# Autodesk Inventor assembly: FemPodstawa
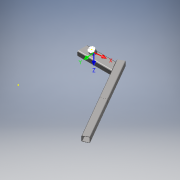
[picture p0: Inventor's stored thumbnail of the model, 180x180]
Saved by Autodesk Inventor 2017 (Build 210142000, 142)
## iProperties
Created: 2016-12-08
Part Number: FemPodstawa
Document SubType Name: Assembly
Designer: Marcin
Author: Marcin
## Documents named in this file (21)
- M:\PracaInżynierska\FEM\FemPodstawa.iam
- M:\PracaInżynierska\PodstawaFem.ipt
- M:\PracaInżynierska\WynikiZadaniaOdwrotnego\PN EN 10219-2 - 100 x 80 x 6  - 655.ipt
- M:\PracaInżynierska\WynikiZadaniaOdwrotnego\PN EN 10219-2 - 160 x 80 x 8  - 545.ipt
- M:\PracaInżynierska\WynikiZadaniaOdwrotnego\PN EN 10060 - 75 - 50.ipt
- M:\PracaInżynierska\WynikiZadaniaOdwrotnego\PN EN 10219-2 - 100 x 80 x 6  - 655_MIR.ipt
- M:\PracaInżynierska\WynikiZadaniaOdwrotnego\PN EN 10219-2 - 160 x 80 x 8  - 545_MIR.ipt
- M:\PracaInżynierska\WynikiZadaniaOdwrotnego\PN EN 10060 - 75 - 50_MIR.ipt
- M:\PracaInżynierska\WynikiZadaniaOdwrotnego\PN EN 10219-2 - 100 x 80 x 6  - 655_MIR1.ipt
- M:\PracaInżynierska\WynikiZadaniaOdwrotnego\PN EN 10219-2 - 160 x 80 x 8  - 545_MIR1.ipt
- M:\PracaInżynierska\WynikiZadaniaOdwrotnego\PN EN 10060 - 75 - 50_MIR1.ipt
- M:\PracaInżynierska\WynikiZadaniaOdwrotnego\PN EN 10219-2 - 100 x 80 x 6  - 655_MIR_MIR.ipt
- M:\PracaInżynierska\WynikiZadaniaOdwrotnego\PN EN 10219-2 - 160 x 80 x 8  - 545_MIR_MIR.ipt
- M:\PracaInżynierska\WynikiZadaniaOdwrotnego\PN EN 10060 - 75 - 50_MIR_MIR.ipt
- M:\PracaInżynierska\PodstawaFem_MIR.ipt
- M:\PracaInżynierska\WynikiZadaniaOdwrotnego\PN EN 10219-2 - 100 x 80 x 6  - 655_MIR2.ipt
- M:\PracaInżynierska\WynikiZadaniaOdwrotnego\PN EN 10219-2 - 160 x 80 x 8  - 545_MIR2.ipt
- M:\PracaInżynierska\WynikiZadaniaOdwrotnego\PN EN 10060 - 75 - 50_MIR2.ipt
- M:\PracaInżynierska\WynikiZadaniaOdwrotnego\PN EN 10219-2 - 100 x 80 x 6  - 655_MIR_MIR1.ipt
- M:\PracaInżynierska\WynikiZadaniaOdwrotnego\PN EN 10219-2 - 160 x 80 x 8  - 545_MIR_MIR1.ipt
- M:\PracaInżynierska\WynikiZadaniaOdwrotnego\PN EN 10060 - 75 - 50_MIR_MIR1.ipt
## Components (20 placed, 20 different names)
1. PodstawaFem:1 — Flush:13
2. PN EN 10219-2 - 100 x 80 x 6  - 655:1 — Mate:3, Flush:5
3. PN EN 10219-2 - 160 x 80 x 8  - 545:1 — Mate:3, Flush:5, Mate:4
4. PodSilownik — Mate:4, Flush:13
5. PN EN 10219-2 - 100 x 80 x 6  - 655_MIR:1 — Flush:6, Mate:5
6. PN EN 10219-2 - 160 x 80 x 8  - 545_MIR:1 — Flush:6, Mate:5, Angle:2, Mate:6
7. PN EN 10060 - 75 - 50_MIR:1 — Angle:2, Mate:6
8. PN EN 10219-2 - 100 x 80 x 6  - 655_MIR1:1 — Flush:7, Mate:7
9. PN EN 10219-2 - 160 x 80 x 8  - 545_MIR1:1 — Flush:7, Mate:7, Angle:3, Mate:8
10. PN EN 10060 - 75 - 50_MIR1:1 — Angle:3, Mate:8
11. PN EN 10219-2 - 100 x 80 x 6  - 655_MIR_MIR:1 — Mate:9, Flush:8
12. PN EN 10219-2 - 160 x 80 x 8  - 545_MIR_MIR:1 — Mate:9, Flush:8, Mate:10, Angle:4
13. PN EN 10060 - 75 - 50_MIR_MIR:1 — Mate:10, Angle:4
14. PodstawaFem_MIR:1
15. PN EN 10219-2 - 100 x 80 x 6  - 655_MIR2:1 — Flush:9, Mate:11
16. PN EN 10219-2 - 160 x 80 x 8  - 545_MIR2:1 — Flush:9, Mate:11, Angle:5, Mate:12
17. PN EN 10060 - 75 - 50_MIR2:1 — Angle:5, Mate:12
18. PN EN 10219-2 - 100 x 80 x 6  - 655_MIR_MIR1:1 — Mate:13, Flush:10
19. PN EN 10219-2 - 160 x 80 x 8  - 545_MIR_MIR1:1 — Mate:13, Flush:10, Mate:14, Angle:6
20. PN EN 10060 - 75 - 50_MIR_MIR1:1 — Mate:14, Angle:6
## Relationships (26: Mate 12, Flush 9, Angle 5)
- Mate:3: PN EN 10219-2 - 100 x 80 x 6  - 655:1 ↔ PN EN 10219-2 - 160 x 80 x 8  - 545:1
- Flush:5: PN EN 10219-2 - 100 x 80 x 6  - 655:1 ↔ PN EN 10219-2 - 160 x 80 x 8  - 545:1
- Mate:4: PN EN 10219-2 - 160 x 80 x 8  - 545:1 ↔ PodSilownik
- Flush:6: PN EN 10219-2 - 100 x 80 x 6  - 655_MIR:1 ↔ PN EN 10219-2 - 160 x 80 x 8  - 545_MIR:1
- Mate:5: PN EN 10219-2 - 100 x 80 x 6  - 655_MIR:1 ↔ PN EN 10219-2 - 160 x 80 x 8  - 545_MIR:1
- Angle:2 (-55 deg): PN EN 10219-2 - 160 x 80 x 8  - 545_MIR:1 ↔ PN EN 10060 - 75 - 50_MIR:1
- Mate:6: PN EN 10219-2 - 160 x 80 x 8  - 545_MIR:1 ↔ PN EN 10060 - 75 - 50_MIR:1
- Flush:7: PN EN 10219-2 - 100 x 80 x 6  - 655_MIR1:1 ↔ PN EN 10219-2 - 160 x 80 x 8  - 545_MIR1:1
- Mate:7: PN EN 10219-2 - 100 x 80 x 6  - 655_MIR1:1 ↔ PN EN 10219-2 - 160 x 80 x 8  - 545_MIR1:1
- Angle:3 (-55 deg): PN EN 10219-2 - 160 x 80 x 8  - 545_MIR1:1 ↔ PN EN 10060 - 75 - 50_MIR1:1
- Mate:8: PN EN 10219-2 - 160 x 80 x 8  - 545_MIR1:1 ↔ PN EN 10060 - 75 - 50_MIR1:1
- Mate:9: PN EN 10219-2 - 100 x 80 x 6  - 655_MIR_MIR:1 ↔ PN EN 10219-2 - 160 x 80 x 8  - 545_MIR_MIR:1
- Flush:8: PN EN 10219-2 - 100 x 80 x 6  - 655_MIR_MIR:1 ↔ PN EN 10219-2 - 160 x 80 x 8  - 545_MIR_MIR:1
- Mate:10: PN EN 10219-2 - 160 x 80 x 8  - 545_MIR_MIR:1 ↔ PN EN 10060 - 75 - 50_MIR_MIR:1
- Angle:4 (55 deg): PN EN 10219-2 - 160 x 80 x 8  - 545_MIR_MIR:1 ↔ PN EN 10060 - 75 - 50_MIR_MIR:1
- Flush:9: PN EN 10219-2 - 100 x 80 x 6  - 655_MIR2:1 ↔ PN EN 10219-2 - 160 x 80 x 8  - 545_MIR2:1
- Mate:11: PN EN 10219-2 - 100 x 80 x 6  - 655_MIR2:1 ↔ PN EN 10219-2 - 160 x 80 x 8  - 545_MIR2:1
- Angle:5 (-55 deg): PN EN 10219-2 - 160 x 80 x 8  - 545_MIR2:1 ↔ PN EN 10060 - 75 - 50_MIR2:1
- Mate:12: PN EN 10219-2 - 160 x 80 x 8  - 545_MIR2:1 ↔ PN EN 10060 - 75 - 50_MIR2:1
- Mate:13: PN EN 10219-2 - 100 x 80 x 6  - 655_MIR_MIR1:1 ↔ PN EN 10219-2 - 160 x 80 x 8  - 545_MIR_MIR1:1
- Flush:10: PN EN 10219-2 - 100 x 80 x 6  - 655_MIR_MIR1:1 ↔ PN EN 10219-2 - 160 x 80 x 8  - 545_MIR_MIR1:1
- Mate:14: PN EN 10219-2 - 160 x 80 x 8  - 545_MIR_MIR1:1 ↔ PN EN 10060 - 75 - 50_MIR_MIR1:1
- Angle:6 (55 deg): PN EN 10219-2 - 160 x 80 x 8  - 545_MIR_MIR1:1 ↔ PN EN 10060 - 75 - 50_MIR_MIR1:1
- [Flush]: PodstawaFem:1 ↔ PodSilownik
- [Flush]: PodstawaFem:1 ↔ PodSilownik
- Flush:13: PodstawaFem:1 ↔ PodSilownik
